# Autodesk Inventor assembly: matriz
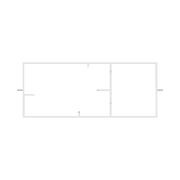
[picture p0: Inventor's stored thumbnail of the model, 180x180]
Saved by Autodesk Inventor 2021 (Build 250183000, 183)
## iProperties
Created: 2021-03-29
Part Number: matriz
Document SubType Name: Assembly
Designer: j2seb
Author: j2seb
## Documents named in this file (4)
- E:\Documentos\Documentos\Michael_Rodriguez\ProyectoAPM\matriz.iam
- E:\Documentos\Documentos\Michael_Rodriguez\Universidad_Nacional\Doceaba_matricula\Automatizacion\Proyecto\Proyecto_APM\02 Inventor\Esqueleto_estructura.ipt
- E:\Documentos\Documentos\Michael_Rodriguez\ProyectoAPM\Pieza2.ipt
- E:\Documentos\Documentos\Michael_Rodriguez\ProyectoAPM\Pieza1.ipt
## Components (4 placed, 3 different names)
1. Esqueleto_estructura:1 — Coincidencia:2, Coincidencia:3, Coincidencia:4, Coincidencia:5, Coincidencia:6, Coincidencia:9, Coincidencia:10
2. Pieza2:1 — Coincidencia:15, Coincidencia:16, Coincidencia:17, Coincidencia:18
3. Pieza1:1 — Coincidencia:15, Coincidencia:17
4. Pieza1:2 — Coincidencia:16, Coincidencia:18
## Relationships (14: Mate 13, Flush 1)
- Coincidencia:2 [Mate]: Esqueleto_estructura:1
- Coincidencia:3 [Mate]: Esqueleto_estructura:1
- Coincidencia:4 [Mate]: Esqueleto_estructura:1
- Coincidencia:5 [Mate]: Esqueleto_estructura:1
- Coincidencia:6 [Mate]: Esqueleto_estructura:1
- Nivelación:3 [Flush] (35 mm)
- Coincidencia:9 [Mate]: Esqueleto_estructura:1
- Coincidencia:10 [Mate]: Esqueleto_estructura:1
- Coincidencia:11 [Mate]
- Coincidencia:13 [Mate]
- Coincidencia:15 [Mate]: Pieza2:1 ↔ Pieza1:1
- Coincidencia:16 [Mate]: Pieza2:1 ↔ Pieza1:2
- Coincidencia:17 [Mate] (-312 mm): Pieza2:1 ↔ Pieza1:1
- Coincidencia:18 [Mate] (-312 mm): Pieza2:1 ↔ Pieza1:2
